# Autodesk Inventor assembly: Leg_joint_roll_yaw
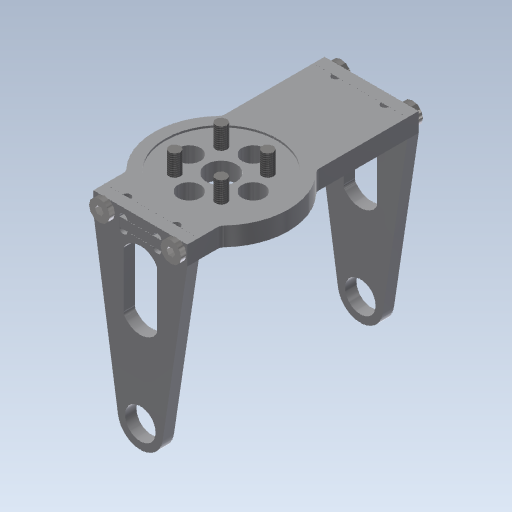
[picture p0: Inventor's stored thumbnail of the model, 512x512]
Saved by Autodesk Inventor 2020.4 (Build 244396000, 396)
## iProperties
Created: 2016-05-01
Part Number: Leg_joint_roll_yaw
Document SubType Name: Assembly
Designer: hiroaki
Mass: 101.489 g
Surface Area: 218.083 cm^2
Volume: 17.9148 cm^3
Density: 5.6651 g/cm^3
Author: hiroaki
## Documents named in this file (5)
- C:\Users\Masato\Documents\Inventor\CIT Brains_Inventor\OpenPlatform_ver3_0 - ver4_1_prototype\LowerBody\Leg_joit\Leg_joint_roll_yaw.iam
- C:\Users\Masato\Documents\Inventor\CIT Brains_Inventor\OpenPlatform_ver3_0 - ver4_1_prototype\LowerBody\Leg_joit\Leg_joint_yaw_frame.ipt
- C:\Users\Masato\Documents\Inventor\CIT Brains_Inventor\OpenPlatform_ver3_0 - ver4_1_prototype\ReadyMade\Screw\M3-10.ipt
- C:\Users\Masato\Documents\Inventor\CIT Brains_Inventor\OpenPlatform_ver3_0 - ver4_1_prototype\LowerBody\Leg_joit\Leg_joint_slider_frame.ipt
- C:\Users\Masato\Documents\Inventor\CIT Brains_Inventor\OpenPlatform_ver3_0 - ver4_1_prototype\ReadyMade\Screw\M3-8.ipt
## Components (11 placed, 4 different names)
1. Leg_joint_yaw_frame:1 — 挿入:1, 挿入:2, 挿入:3, 挿入:4, 挿入:5, 挿入:6, 挿入:7, 挿入:8, フラッシュ:1, フラッシュ:2, メイト:1
2. Leg_joint_slider_frame:1 — 挿入:1, 挿入:2, 挿入:77, 挿入:78
3. Leg_joint_slider_frame:2 — 挿入:3, 挿入:4, 挿入:79, 挿入:80
4. M3-8:4 — 挿入:80
5. M3-8:3 — 挿入:79
6. M3-8:2 — 挿入:78
7. M3-8:1 — 挿入:77
8. M3-10:4 — 挿入:8
9. M3-10:3 — 挿入:7
10. M3-10:2 — 挿入:6
11. M3-10:1 — 挿入:5
## Relationships (15: Insert 12, Flush 2, Mate 1)
- 挿入:1 [Insert]: Leg_joint_yaw_frame:1 ↔ Leg_joint_slider_frame:1
- 挿入:2 [Insert]: Leg_joint_yaw_frame:1 ↔ Leg_joint_slider_frame:1
- 挿入:3 [Insert]: Leg_joint_yaw_frame:1 ↔ Leg_joint_slider_frame:2
- 挿入:4 [Insert]: Leg_joint_yaw_frame:1 ↔ Leg_joint_slider_frame:2
- 挿入:5 [Insert]: Leg_joint_yaw_frame:1 ↔ M3-10:1
- 挿入:6 [Insert]: Leg_joint_yaw_frame:1 ↔ M3-10:2
- 挿入:7 [Insert]: Leg_joint_yaw_frame:1 ↔ M3-10:3
- 挿入:8 [Insert]: Leg_joint_yaw_frame:1 ↔ M3-10:4
- フラッシュ:1 [Flush]: Leg_joint_yaw_frame:1
- フラッシュ:2 [Flush]: Leg_joint_yaw_frame:1
- メイト:1 [Mate]: Leg_joint_yaw_frame:1
- 挿入:77 [Insert]: Leg_joint_slider_frame:1 ↔ M3-8:1
- 挿入:78 [Insert]: Leg_joint_slider_frame:1 ↔ M3-8:2
- 挿入:79 [Insert]: Leg_joint_slider_frame:2 ↔ M3-8:3
- 挿入:80 [Insert]: Leg_joint_slider_frame:2 ↔ M3-8:4
